# Autodesk Inventor assembly: Assembly1
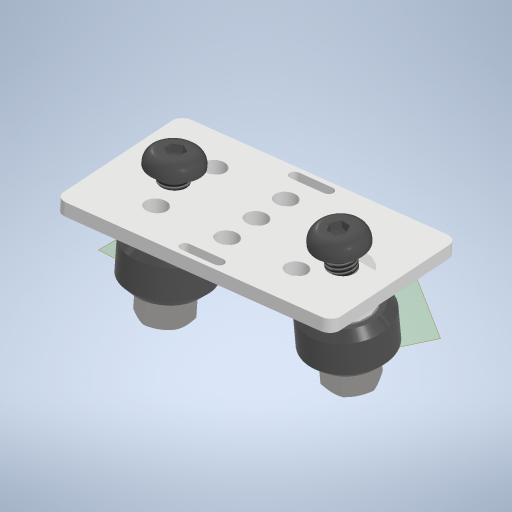
[picture p0: Inventor's stored thumbnail of the model, 512x512]
Saved by Autodesk Inventor 2024 (Build 280153000, 153)
## iProperties
Created: 2024-12-08
Part Number: Assembly1
Document SubType Name: Assembly
Designer: Nada
Author: Nada
## Documents named in this file (3)
- C:\Users\Adham\Desktop\Modelling Project\Modeling model\Modeling model\Assembly1.iam
- C:\Users\Adham\Desktop\Modelling Project\Modeling model\Modeling model\Cart.ipt
- C:\Users\Adham\Desktop\Modelling Project\Modeling model\Modeling model\Delrin Mini V-Wheel.iam
## Components (3 placed, 2 different names)
1. Cart:1 — Insert:1
2. Delrin Mini V-Wheel:1 [sub-assembly]
3. Delrin Mini V-Wheel:2 [sub-assembly] — Insert:1
## Relationships (1: Insert 1)
- Insert:1: Cart:1 ↔ Delrin Mini V-Wheel:2
